# Autodesk Inventor assembly: AgarMouldAssembly
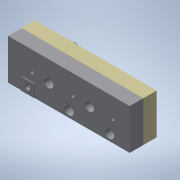
[picture p0: Inventor's stored thumbnail of the model, 180x180]
Saved by Autodesk Inventor 2022 (Build 260153000, 153)
## iProperties
Created: 2016-01-19
Part Number: AgarMouldAssembly
Document SubType Name: Assembly
Designer: 120pa
Author: 120pa
## Documents named in this file (6)
- C:\Users\Spectral\Documents\GitHub\manuscripts\2016-welf-meSPIM\AgarMouldAssembly.iam
- C:\Users\Spectral\Documents\GitHub\manuscripts\2016-welf-meSPIM\AgarMouldBottomV3.ipt
- C:\Users\Spectral\Documents\GitHub\manuscripts\2016-welf-meSPIM\AgarMould.ipt
- C:\Users\Spectral\Documents\GitHub\manuscripts\2016-welf-meSPIM\boltV5.ipt
- C:\Users\Spectral\Documents\GitHub\manuscripts\2016-welf-meSPIM\AgarHolderPEEK_v4.ipt
- C:\Users\Spectral\Documents\GitHub\CAD\Multiscale\sample_holder\agarose_mount.ipt
## Components (5 placed, 5 different names)
1. AgarMouldBottomV3:1 — Mate:1, Flush:1, Flush:2, Mate:2, Mate:3, Mate:4, Mate:5
2. AgarMould:1 — Mate:1, Flush:1, Flush:2, Angle:1, Angle:2
3. boltV5:1 — Angle:1, Mate:2
4. AgarHolderPEEK_v4:1 — Mate:3
5. agarose_mount:1 — Mate:4, Angle:2, Mate:5
## Relationships (9: Mate 5, Flush 2, Angle 2)
- Mate:1: AgarMouldBottomV3:1 ↔ AgarMould:1
- Flush:1: AgarMouldBottomV3:1 ↔ AgarMould:1
- Flush:2: AgarMouldBottomV3:1 ↔ AgarMould:1
- Angle:1 (90 deg): AgarMould:1 ↔ boltV5:1
- Mate:2: AgarMouldBottomV3:1 ↔ boltV5:1
- Mate:3: AgarMouldBottomV3:1 ↔ AgarHolderPEEK_v4:1
- Mate:4: AgarMouldBottomV3:1 ↔ agarose_mount:1
- Angle:2 (0 deg): AgarMould:1 ↔ agarose_mount:1
- Mate:5: AgarMouldBottomV3:1 ↔ agarose_mount:1
